# Autodesk Inventor assembly: SBR16UU
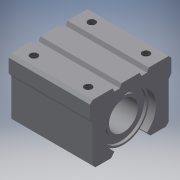
[picture p0: Inventor's stored thumbnail of the model, 180x180]
Saved by Autodesk Inventor 2018 (Build 220112000, 112)
## iProperties
Created: 2018-09-20
Part Number: SBR16UU
Material: Genérico
Document SubType Name: Assembly
Designer: Georgines
Author: Georgines
## Documents named in this file (4)
- C:\Users\Georgines\Documents\EstacaoBGA\Peças 3D\SBR16UU.iam
- C:\Users\Georgines\Documents\EstacaoBGA\Peças 3D\PilowBlockAbertoSBR16.ipt
- C:\Users\Georgines\Documents\EstacaoBGA\Peças 3D\rolamento_linear_lm16uu.iam.ipt
- rolamento_linear_lm16uu.iam
## Components (2 placed, 2 different names)
1. PilowBlockAbertoSBR16:2 — Alinhamento:1
2. rolamento_linear_lm16uu.iam:1 — Alinhamento:1
## Relationships (1: Flush 1)
- Alinhamento:1 [Flush] (4 mm): PilowBlockAbertoSBR16:2 ↔ rolamento_linear_lm16uu.iam:1
